# Autodesk Inventor assembly: Base_Assembly
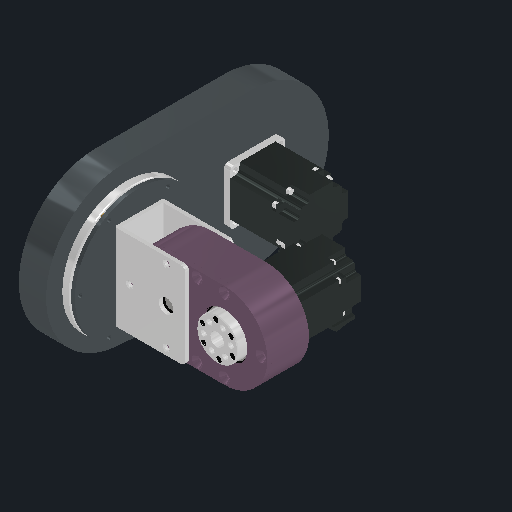
[picture p0: Inventor's stored thumbnail of the model, 512x512]
Saved by Autodesk Inventor 2026 (Build 300175000, 175)
## iProperties
RuleStatus: InUse
Created: 2025-11-30
Part Number: Base_Assembly
Document SubType Name: Assembly
Designer: pochi
Mass: 2736.74 g
Surface Area: 4914.19 cm^2
Volume: 1577.66 cm^3
Density: 1.73469 g/cm^3
Author: pochi
## Documents named in this file (13)
- D:\POLIMI\3RD SEMESTER\Industrial Robotics\Project\Mine\Base_Assembly.iam
- D:\POLIMI\3RD SEMESTER\Industrial Robotics\Project\Mine\BASE.ipt
- D:\POLIMI\3RD SEMESTER\Industrial Robotics\Project\Mine\TurnableBearing.ipt
- D:\POLIMI\3RD SEMESTER\Industrial Robotics\Project\Mine\Spacer_05.ipt
- D:\POLIMI\3RD SEMESTER\Industrial Robotics\Project\Mine\Plate.ipt
- D:\POLIMI\3RD SEMESTER\Industrial Robotics\Project\Mine\Fold.ipt
- D:\POLIMI\3RD SEMESTER\Industrial Robotics\Project\Mine\FlangeHub.ipt
- D:\POLIMI\3RD SEMESTER\Industrial Robotics\Project\Mine\Shaft_02.ipt
- D:\POLIMI\3RD SEMESTER\Industrial Robotics\Project\Mine\3M120T.ipt
- D:\POLIMI\3RD SEMESTER\Industrial Robotics\Project\Mine\3M120T_03.ipt
- D:\POLIMI\3RD SEMESTER\Industrial Robotics\Project\Mine\Belt_03.ipt
- D:\POLIMI\3RD SEMESTER\Industrial Robotics\Project\Mine\Reducer.iam
- D:\POLIMI\3RD SEMESTER\Industrial Robotics\Project\Mine\Motor_02.ipt
## Components (23 placed, 12 different names)
1. BASE:1 — Mate:1, Mate:2, Mate:3, Mate:4, Mate:5, Mate:6, Mate:7, Mate:9, Mate:10, Mate:37, Mate:44, Mate:45
2. TurnableBearing:1 — Mate:1, Mate:2, Mate:11, Mate:12, Mate:13, Mate:14, Mate:15, Mate:16, Mate:17, Mate:18, Mate:19, Mate:20, Mate:21, Mate:22, Mate:23, Mate:24
3. Spacer_05:1 — Mate:9, Flush:5
4. Spacer_05:2 — Flush:2, Mate:7, Flush:4, Flush:5
5. Spacer_05:3 — Mate:3, Mate:4, Flush:1, Flush:2, Flush:3, Mate:11
6. Spacer_05:4 — Flush:1, Mate:5
7. Spacer_05:5 — Flush:3, Mate:6
8. Spacer_05:6 — Flush:4, Mate:10
9. Spacer_05:7 — Mate:12, Mate:13
10. Spacer_05:8 — Mate:18, Mate:19
11. Spacer_05:9 — Mate:16, Mate:20, Mate:25, Mate:26
12. Spacer_05:10 — Mate:17, Mate:21
13. Spacer_05:11 — Mate:14, Mate:23
14. Spacer_05:12 — Mate:15, Mate:22
15. Plate:1 — Mate:24, Mate:25, Mate:26, Mate:27, Mate:28, Mate:29, Mate:30, Mate:31, Mate:32, Mate:33
16. Fold:1 — Mate:27, Mate:28, Mate:29, Mate:41, Mate:42, Mate:43
17. FlangeHub:1 — Mate:30, Mate:31, Mate:32, Mate:34, Mate:35
18. Shaft_02:1 — Mate:33, Mate:34, Mate:36
19. 3M120T:1 — Mate:35, Mate:36, Flush:6, Mate:38
20. 3M120T_03:1 — Mate:37, Flush:6, Mate:39, Mate:40
21. Belt_03:1 — Mate:38, Mate:39, Mate:40
22. Reducer:1 [sub-assembly] — Mate:41, Mate:42, Mate:43
23. Motor_02:1 — Mate:44, Mate:45
## Relationships (50: Mate 44, Flush 6)
- Mate:1: BASE:1 ↔ TurnableBearing:1
- Mate:2: BASE:1 ↔ TurnableBearing:1
- Mate:3: BASE:1 ↔ Spacer_05:3
- Mate:4: BASE:1 ↔ Spacer_05:3
- Flush:1: Spacer_05:3 ↔ Spacer_05:4
- Flush:2: Spacer_05:2 ↔ Spacer_05:3
- Flush:3: Spacer_05:3 ↔ Spacer_05:5
- Mate:5: BASE:1 ↔ Spacer_05:4
- Mate:6: BASE:1 ↔ Spacer_05:5
- Mate:7: BASE:1 ↔ Spacer_05:2
- Mate:9: BASE:1 ↔ Spacer_05:1
- Flush:4: Spacer_05:2 ↔ Spacer_05:6
- Mate:10: BASE:1 ↔ Spacer_05:6
- Flush:5: Spacer_05:1 ↔ Spacer_05:2
- Mate:11: TurnableBearing:1 ↔ Spacer_05:3
- Mate:12: TurnableBearing:1 ↔ Spacer_05:7
- Mate:13: TurnableBearing:1 ↔ Spacer_05:7
- Mate:14: TurnableBearing:1 ↔ Spacer_05:11
- Mate:15: TurnableBearing:1 ↔ Spacer_05:12
- Mate:16: TurnableBearing:1 ↔ Spacer_05:9
- Mate:17: TurnableBearing:1 ↔ Spacer_05:10
- Mate:18: TurnableBearing:1 ↔ Spacer_05:8
- Mate:19: TurnableBearing:1 ↔ Spacer_05:8
- Mate:20: TurnableBearing:1 ↔ Spacer_05:9
- Mate:21: TurnableBearing:1 ↔ Spacer_05:10
- Mate:22: TurnableBearing:1 ↔ Spacer_05:12
- Mate:23: TurnableBearing:1 ↔ Spacer_05:11
- Mate:24: TurnableBearing:1 ↔ Plate:1
- Mate:25: Spacer_05:9 ↔ Plate:1
- Mate:26: Spacer_05:9 ↔ Plate:1
- Mate:27: Plate:1 ↔ Fold:1
- Mate:28: Plate:1 ↔ Fold:1
- Mate:29: Plate:1 ↔ Fold:1
- Mate:30: Plate:1 ↔ FlangeHub:1
- Mate:31: Plate:1 ↔ FlangeHub:1
- Mate:32: Plate:1 ↔ FlangeHub:1
- Mate:33: Plate:1 ↔ Shaft_02:1
- Mate:34: FlangeHub:1 ↔ Shaft_02:1
- Mate:35 (2 mm): FlangeHub:1 ↔ 3M120T:1
- Mate:36: Shaft_02:1 ↔ 3M120T:1
- Mate:37: BASE:1 ↔ 3M120T_03:1
- Flush:6: 3M120T:1 ↔ 3M120T_03:1
- Mate:38: 3M120T:1 ↔ Belt_03:1
- Mate:39: 3M120T_03:1 ↔ Belt_03:1
- Mate:40: 3M120T_03:1 ↔ Belt_03:1
- Mate:41: Fold:1 ↔ Reducer:1
- Mate:42: Fold:1 ↔ Reducer:1
- Mate:43: Fold:1 ↔ Reducer:1
- Mate:44: BASE:1 ↔ Motor_02:1
- Mate:45: BASE:1 ↔ Motor_02:1
